# Autodesk Inventor assembly: Fulle Assembly
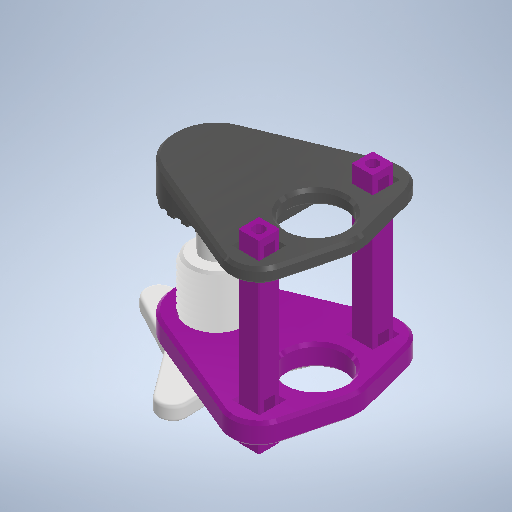
[picture p0: Inventor's stored thumbnail of the model, 512x512]
Saved by Autodesk Inventor 2026.2 (Build 302298010, 298A)
## iProperties
Created: 2026-05-07
Part Number: Fulle Assembly
Document SubType Name: Assembly
Designer: piete
Author: piete
## Documents named in this file (6)
- C:\Users\piete\Desktop\Skripsie\Documents\Detail Design\Arm Design\Fulle Assembly.iam
- C:\Users\piete\Desktop\Skripsie\Documents\Detail Design\Arm Design\Bottom Clamp\Bottom Frame.ipt
- C:\Users\piete\Desktop\Skripsie\Documents\Detail Design\Arm Design\Bottom Clamp\Top Frame.ipt
- C:\Users\piete\Desktop\Skripsie\Documents\Detail Design\Arm Design\Bottom Clamp\Power Screw.ipt
- C:\Users\piete\Desktop\Skripsie\Documents\Detail Design\Arm Design\Bottom Clamp\Foot Stamp.ipt
- C:\Users\piete\Desktop\Skripsie\Documents\Detail Design\Arm Design\Bottom Clamp\Square Supports.ipt
## Components (6 placed, 5 different names)
1. Bottom Frame:1 — Flush:1, Flush:2, Mate:1, Mate:2, Mate:4, Mate:5, Mate:6, Mate:7, Mate:8, Mate:9, Mate:10
2. Top Frame:1 — Flush:1, Flush:2, Mate:4
3. Power Screw:1 — Mate:1, Mate:2, Mate:3, Flush:3, Flush:4
4. Foot Stamp:1 — Mate:3, Flush:3, Flush:4
5. Square Supports:1 — Mate:5, Mate:6, Mate:7
6. Square Supports:2 — Mate:8, Mate:9, Mate:10
## Relationships (14: Mate 10, Flush 4)
- Flush:1: Bottom Frame:1 ↔ Top Frame:1
- Flush:2: Bottom Frame:1 ↔ Top Frame:1
- Mate:1: Bottom Frame:1 ↔ Power Screw:1
- Mate:2 (10 mm): Bottom Frame:1 ↔ Power Screw:1
- Mate:3: Power Screw:1 ↔ Foot Stamp:1
- Flush:3: Power Screw:1 ↔ Foot Stamp:1
- Flush:4: Power Screw:1 ↔ Foot Stamp:1
- Mate:4 (70 mm): Bottom Frame:1 ↔ Top Frame:1
- Mate:5 (0.1 mm): Bottom Frame:1 ↔ Square Supports:1
- Mate:6 (0.1 mm): Bottom Frame:1 ↔ Square Supports:1
- Mate:7 (5 mm): Bottom Frame:1 ↔ Square Supports:1
- Mate:8: Bottom Frame:1 ↔ Square Supports:2
- Mate:9 (5 mm): Bottom Frame:1 ↔ Square Supports:2
- Mate:10 (0.1 mm): Bottom Frame:1 ↔ Square Supports:2
